# Autodesk Inventor assembly: AssemblyfinalRRPR
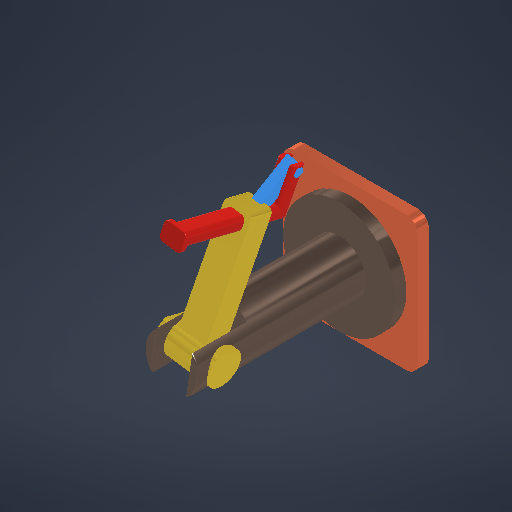
[picture p0: Inventor's stored thumbnail of the model, 512x512]
Saved by Autodesk Inventor 2026 (Build 300175050, 175E)
## iProperties
Created: 2026-05-06
Part Number: AssemblyfinalRRPR
Document SubType Name: Assembly
Designer: ptp527
Author: ptp527
## Documents named in this file (6)
- H:\Inventor\Kinematics\finalkinematic\AssemblyfinalRRPR.iam
- H:\Inventor\Kinematics\finalkinematic\Part1final.ipt
- H:\Inventor\Kinematics\finalkinematic\Part2final.ipt
- H:\Inventor\Kinematics\finalkinematic\Part3final.ipt
- H:\Inventor\Kinematics\finalkinematic\Part4final.ipt
- H:\Inventor\Kinematics\finalkinematic\Part1Grroundfinal.ipt
## Components (5 placed, 5 different names)
1. Part1final:1 — Rotational:1, Rotational:3
2. Part2final:1 — Rotational:1, Slider:1
3. Part3final:1 — Slider:1, Rotational:2
4. Part4final:1 — Rotational:2
5. Part1Grroundfinal:1 — Rotational:3
## Relationships (4: RevoluteJoint 3, TranslationJoint 1)
- Rotational:1 [RevoluteJoint]: Part1final:1 ↔ Part2final:1
- Slider:1 [TranslationJoint]: Part2final:1 ↔ Part3final:1
- Rotational:2 [RevoluteJoint]: Part3final:1 ↔ Part4final:1
- Rotational:3 [RevoluteJoint]: Part1final:1 ↔ Part1Grroundfinal:1
